# Autodesk Inventor assembly: Intake Full Assembly
(part 2 of 2)
- Mate:580: Intake Roller Plate:1 ↔ COTS_92949A265_1-2in long Stainless Steel Button Head Screw:19
- Mate:581: Intake Roller Plate:1 ↔ COTS_92949A265_1-2in long Stainless Steel Button Head Screw:21
- Mate:582: Intake Roller Plate:1 ↔ COTS_92949A265_1-2in long Stainless Steel Button Head Screw:9
- Mate:583: Intake Roller Plate:1 ↔ COTS_92949A265_1-2in long Stainless Steel Button Head Screw:9
- Mate:584: Intake Roller Plate:1 ↔ COTS_92949A265_1-2in long Stainless Steel Button Head Screw:21
- Mate:585: Intake Roller Plate:1 ↔ COTS_92949A265_1-2in long Stainless Steel Button Head Screw:19
- Mate:586: Intake Roller Plate:1 ↔ COTS_92949A265_1-2in long Stainless Steel Button Head Screw:6
- Mate:587: Intake Roller Plate:1 ↔ COTS_92949A265_1-2in long Stainless Steel Button Head Screw:20
- Mate:588: Intake Roller Plate:1 ↔ COTS_92949A265_1-2in long Stainless Steel Button Head Screw:8
- Mate:589: INTK_001_PulleyCover:1 ↔ COTS_92949A265_1-2in long Stainless Steel Button Head Screw:14
- Mate:590: INTK_001_PulleyCover:1 ↔ COTS_92949A265_1-2in long Stainless Steel Button Head Screw:15
- Mate:591: INTK_001_PulleyCover:1 ↔ COTS_92949A265_1-2in long Stainless Steel Button Head Screw:24
- Mate:592: INTK_001_PulleyCover:1 ↔ COTS_92949A265_1-2in long Stainless Steel Button Head Screw:17
- Mate:593: INTK_001_PulleyCover:1 ↔ COTS_92949A265_1-2in long Stainless Steel Button Head Screw:18
- Mate:594: INTK_001_PulleyCover:1 ↔ COTS_92949A265_1-2in long Stainless Steel Button Head Screw:7
- Mate:595: INTK_001_PulleyCover:1 ↔ COTS_92949A265_1-2in long Stainless Steel Button Head Screw:16
- Mate:596: INTK_001_PulleyCover:2 ↔ COTS_92949A265_1-2in long Stainless Steel Button Head Screw:2
- Mate:597: INTK_001_PulleyCover:2 ↔ COTS_92949A265_1-2in long Stainless Steel Button Head Screw:5
- Mate:598: INTK_001_PulleyCover:2 ↔ COTS_92949A265_1-2in long Stainless Steel Button Head Screw:4
- Mate:599: INTK_001_PulleyCover:2 ↔ COTS_92949A265_1-2in long Stainless Steel Button Head Screw:1
- Mate:600: INTK_001_PulleyCover:2 ↔ COTS_92949A265_1-2in long Stainless Steel Button Head Screw:12
- Mate:601: INTK_001_PulleyCover:2 ↔ COTS_92949A265_1-2in long Stainless Steel Button Head Screw:13
- Mate:602: INTK_001_PulleyCover:2 ↔ COTS_92949A265_1-2in long Stainless Steel Button Head Screw:3
- Mate:603: INTK_001_PulleyCover:2 ↔ COTS_92949A265_1-2in long Stainless Steel Button Head Screw:13
- Mate:604: INTK_001_PulleyCover:2 ↔ COTS_92949A265_1-2in long Stainless Steel Button Head Screw:3
- Mate:605: INTK_001_PulleyCover:2 ↔ COTS_92949A265_1-2in long Stainless Steel Button Head Screw:1
- Mate:606: INTK_001_PulleyCover:2 ↔ COTS_92949A265_1-2in long Stainless Steel Button Head Screw:2
- Mate:607: INTK_001_PulleyCover:2 ↔ COTS_92949A265_1-2in long Stainless Steel Button Head Screw:5
- Mate:608: INTK_001_PulleyCover:2 ↔ COTS_92949A265_1-2in long Stainless Steel Button Head Screw:4
- Mate:609: INTK_001_PulleyCover:2 ↔ COTS_92949A265_1-2in long Stainless Steel Button Head Screw:12
- Mate:610: Intake Roller Plate:2 ↔ COTS_92949A265_1-2in long Stainless Steel Button Head Screw:26
- Mate:611: Intake Roller Plate:2 ↔ COTS_92949A265_1-2in long Stainless Steel Button Head Screw:11
- Mate:612: Intake Roller Plate:2 ↔ COTS_92949A265_1-2in long Stainless Steel Button Head Screw:25
- Mate:613: Intake Roller Plate:2 ↔ COTS_92949A265_1-2in long Stainless Steel Button Head Screw:27
- Mate:614: Intake Roller Plate:2 ↔ COTS_92949A265_1-2in long Stainless Steel Button Head Screw:23
- Mate:615: Intake Roller Plate:2 ↔ COTS_92949A265_1-2in long Stainless Steel Button Head Screw:22
- Mate:616: Intake Roller Plate:2 ↔ COTS_92949A265_1-2in long Stainless Steel Button Head Screw:26
- Mate:617: Intake Roller Plate:2 ↔ COTS_92949A265_1-2in long Stainless Steel Button Head Screw:22
- Mate:618: Intake Roller Plate:2 ↔ COTS_92949A265_1-2in long Stainless Steel Button Head Screw:23
- Mate:619: Intake Roller Plate:2 ↔ COTS_92949A265_1-2in long Stainless Steel Button Head Screw:27
- Mate:620: Intake Roller Plate:2 ↔ COTS_92949A265_1-2in long Stainless Steel Button Head Screw:25
- Mate:621: Intake Roller Plate:2 ↔ COTS_92949A265_1-2in long Stainless Steel Button Head Screw:11
- Mate:622: COTS_217-2592_VersaHub:2 ↔ COTS_91251A196_Black-Oxide Alloy Steel Socket Head Screw_5-8in:3
- Mate:623: COTS_217-2592_VersaHub:2 ↔ COTS_91251A196_Black-Oxide Alloy Steel Socket Head Screw_5-8in:1
- Mate:624: COTS_217-2592_VersaHub:2 ↔ COTS_91251A196_Black-Oxide Alloy Steel Socket Head Screw_5-8in:2
- Mate:625: COTS_217-2592_VersaHub:2 ↔ COTS_91251A196_Black-Oxide Alloy Steel Socket Head Screw_5-8in:11
- Mate:626: COTS_217-2592_VersaHub:2 ↔ COTS_91251A196_Black-Oxide Alloy Steel Socket Head Screw_5-8in:4
- Mate:627: COTS_217-2592_VersaHub:2 ↔ COTS_91251A196_Black-Oxide Alloy Steel Socket Head Screw_5-8in:6
- Mate:628: COTS_217-2592_VersaHub:2 ↔ COTS_91251A196_Black-Oxide Alloy Steel Socket Head Screw_5-8in:4
- Mate:629: COTS_217-2592_VersaHub:2 ↔ COTS_91251A196_Black-Oxide Alloy Steel Socket Head Screw_5-8in:6
- Mate:630: COTS_217-2592_VersaHub:2 ↔ COTS_91251A196_Black-Oxide Alloy Steel Socket Head Screw_5-8in:11
- Mate:631: COTS_217-2592_VersaHub:2 ↔ COTS_91251A196_Black-Oxide Alloy Steel Socket Head Screw_5-8in:2
- Mate:632: COTS_217-2592_VersaHub:2 ↔ COTS_91251A196_Black-Oxide Alloy Steel Socket Head Screw_5-8in:3
- Mate:633: COTS_217-2592_VersaHub:2 ↔ COTS_91251A196_Black-Oxide Alloy Steel Socket Head Screw_5-8in:1
- Mate:634: COTS_217-2592_VersaHub:3 ↔ COTS_91251A196_Black-Oxide Alloy Steel Socket Head Screw_5-8in:12
- Mate:635: COTS_217-2592_VersaHub:3 ↔ COTS_91251A196_Black-Oxide Alloy Steel Socket Head Screw_5-8in:7
- Mate:636: COTS_217-2592_VersaHub:3 ↔ COTS_91251A196_Black-Oxide Alloy Steel Socket Head Screw_5-8in:10
- Mate:637: COTS_217-2592_VersaHub:3 ↔ COTS_91251A196_Black-Oxide Alloy Steel Socket Head Screw_5-8in:9
- Mate:638: COTS_217-2592_VersaHub:3 ↔ COTS_91251A196_Black-Oxide Alloy Steel Socket Head Screw_5-8in:5
- Mate:639: COTS_217-2592_VersaHub:3 ↔ COTS_91251A196_Black-Oxide Alloy Steel Socket Head Screw_5-8in:8
- Mate:640: COTS_217-2592_VersaHub:3 ↔ COTS_91251A196_Black-Oxide Alloy Steel Socket Head Screw_5-8in:12
- Mate:641: COTS_217-2592_VersaHub:3 ↔ COTS_91251A196_Black-Oxide Alloy Steel Socket Head Screw_5-8in:7
- Mate:642: COTS_217-2592_VersaHub:3 ↔ COTS_91251A196_Black-Oxide Alloy Steel Socket Head Screw_5-8in:10
- Mate:643: COTS_217-2592_VersaHub:3 ↔ COTS_91251A196_Black-Oxide Alloy Steel Socket Head Screw_5-8in:8
- Mate:644: COTS_217-2592_VersaHub:3 ↔ COTS_91251A196_Black-Oxide Alloy Steel Socket Head Screw_5-8in:5
- Mate:645: COTS_217-2592_VersaHub:3 ↔ COTS_91251A196_Black-Oxide Alloy Steel Socket Head Screw_5-8in:9
- Mate:646: COTS_91251A196_Black-Oxide Alloy Steel Socket Head Screw_5-8in:10 ↔ COTS_90631A009_8-32_Low-Strength Steel Nylon-Insert Locknut:11
- Mate:647: Intake Roller Plate:2 ↔ COTS_90631A009_8-32_Low-Strength Steel Nylon-Insert Locknut:11
- Mate:648: COTS_91251A196_Black-Oxide Alloy Steel Socket Head Screw_5-8in:8 ↔ COTS_90631A009_8-32_Low-Strength Steel Nylon-Insert Locknut:1
- Mate:649: Intake Roller Plate:2 ↔ COTS_90631A009_8-32_Low-Strength Steel Nylon-Insert Locknut:1
- Mate:650: COTS_91251A196_Black-Oxide Alloy Steel Socket Head Screw_5-8in:7 ↔ COTS_90631A009_8-32_Low-Strength Steel Nylon-Insert Locknut:12
- Mate:651: Intake Roller Plate:2 ↔ COTS_90631A009_8-32_Low-Strength Steel Nylon-Insert Locknut:12
- Mate:652: COTS_91251A196_Black-Oxide Alloy Steel Socket Head Screw_5-8in:12 ↔ COTS_90631A009_8-32_Low-Strength Steel Nylon-Insert Locknut:4
- Mate:653: Intake Roller Plate:2 ↔ COTS_90631A009_8-32_Low-Strength Steel Nylon-Insert Locknut:4
- Mate:654: COTS_91251A196_Black-Oxide Alloy Steel Socket Head Screw_5-8in:5 ↔ COTS_90631A009_8-32_Low-Strength Steel Nylon-Insert Locknut:8
- Mate:655: Intake Roller Plate:2 ↔ COTS_90631A009_8-32_Low-Strength Steel Nylon-Insert Locknut:8
- Mate:656: COTS_91251A196_Black-Oxide Alloy Steel Socket Head Screw_5-8in:9 ↔ COTS_90631A009_8-32_Low-Strength Steel Nylon-Insert Locknut:7
- Mate:657: Intake Roller Plate:2 ↔ COTS_90631A009_8-32_Low-Strength Steel Nylon-Insert Locknut:7
- Mate:658: COTS_91251A196_Black-Oxide Alloy Steel Socket Head Screw_5-8in:3 ↔ COTS_90631A009_8-32_Low-Strength Steel Nylon-Insert Locknut:5
- Mate:659: COTS_91251A196_Black-Oxide Alloy Steel Socket Head Screw_5-8in:2 ↔ COTS_90631A009_8-32_Low-Strength Steel Nylon-Insert Locknut:9
- Mate:660: COTS_91251A196_Black-Oxide Alloy Steel Socket Head Screw_5-8in:4 ↔ COTS_90631A009_8-32_Low-Strength Steel Nylon-Insert Locknut:10
- Mate:661: COTS_91251A196_Black-Oxide Alloy Steel Socket Head Screw_5-8in:6 ↔ COTS_90631A009_8-32_Low-Strength Steel Nylon-Insert Locknut:6
- Mate:662: COTS_91251A196_Black-Oxide Alloy Steel Socket Head Screw_5-8in:11 ↔ COTS_90631A009_8-32_Low-Strength Steel Nylon-Insert Locknut:2
- Mate:663: COTS_91251A196_Black-Oxide Alloy Steel Socket Head Screw_5-8in:1 ↔ COTS_90631A009_8-32_Low-Strength Steel Nylon-Insert Locknut:3
- Mate:664: Intake Roller Plate:1 ↔ COTS_90631A009_8-32_Low-Strength Steel Nylon-Insert Locknut:3
- Mate:665: Intake Roller Plate:1 ↔ COTS_90631A009_8-32_Low-Strength Steel Nylon-Insert Locknut:5
- Mate:666: Intake Roller Plate:1 ↔ COTS_90631A009_8-32_Low-Strength Steel Nylon-Insert Locknut:9
- Mate:667: Intake Roller Plate:1 ↔ COTS_90631A009_8-32_Low-Strength Steel Nylon-Insert Locknut:10
- Mate:668: Intake Roller Plate:1 ↔ COTS_90631A009_8-32_Low-Strength Steel Nylon-Insert Locknut:6
- Mate:669: Intake Roller Plate:1 ↔ COTS_90631A009_8-32_Low-Strength Steel Nylon-Insert Locknut:2
- Mate:670: Intake Roller Plate:1 ↔ COTS_92949A265_1-2in long Stainless Steel Button Head Screw:28
- Mate:674: Intake Roller Plate:1 ↔ COTS_92949A265_1-2in long Stainless Steel Button Head Screw:28
- Mate:675: COTS_WCP-0783_1.125ODHexBearing:19 ↔ INtk_010_Belt2:1
- Mate:676 (0.508 mm): COTS_WCP-0783_1.125ODHexBearing:14 ↔ INtk_010_Belt2:1
- Mate:677: COTS_HTD5M10mm15T_WCP-1420:4 ↔ INtk_010_Belt2:1
- Mate:678: COTS_WCP-0783_1.125ODHexBearing:14 ↔ INTK_009_Belt1:1
- Mate:679: INTK_006_Spacer6:1 ↔ INTK_009_Belt1:1
- Mate:680: COTW_HTD5M10mm12T_WCP-0076:1 ↔ INTK_009_Belt1:1
- Mate:681: COTS_WCP-0783_1.125ODHexBearing:20 ↔ INtk_010_Belt2:2
- Mate:682: COTS_WCP-0783_1.125ODHexBearing:15 ↔ INtk_010_Belt2:2
- Mate:683: COTS_HTD5M10mm15T_WCP-1420:1 ↔ INtk_010_Belt2:2
- Mate:684: COTS_WCP-0799_0.5inchHexShaftCollar:8 ↔ INTK_011_Belt3:1
- Mate:685: COTS_WCP-0799_0.5inchHexShaftCollar:7 ↔ INTK_011_Belt3:1
- Mate:686: COTS_HTD5M10mm18T_WCP-0563:18 ↔ INTK_011_Belt3:1
- Mate:687: COTS_WCP-0799_0.5inchHexShaftCollar:6 ↔ INTK_011_Belt3:2
- Mate:688: COTS_WCP-0799_0.5inchHexShaftCollar:5 ↔ INTK_011_Belt3:2
- Mate:689: COTS_HTD5M10mm18T_WCP-0563:5 ↔ INTK_011_Belt3:2
- Mate:690: COTS_WCP-0799_0.5inchHexShaftCollar:11 ↔ INTK_012_Belt4:1
- Mate:691: COTS_WCP-0799_0.5inchHexShaftCollar:9 ↔ INTK_012_Belt4:1
- Mate:692: COTS_HTD5M10mm18T_WCP-0563:4 ↔ INTK_012_Belt4:1
- Mate:693: COTS_WCP-0799_0.5inchHexShaftCollar:10 ↔ INTK_012_Belt4:2
- Mate:694: COTS_WCP-0799_0.5inchHexShaftCollar:12 ↔ INTK_012_Belt4:2
- Mate:695: Intake Roller Plate:2 ↔ INTK_012_Belt4:2
- Mate:696: INTK_005_Spacer5:6 ↔ INTK_013_Belt5:1
- Mate:697: INTK_005_Spacer5:7 ↔ INTK_013_Belt5:1
- Mate:698: COTS_HTD5M10mm18T_WCP-0563:15 ↔ INTK_013_Belt5:1
- Mate:699: INTK_005_Spacer5:4 ↔ INTK_013_Belt5:2
- Mate:700: INTK_005_Spacer5:2 ↔ INTK_013_Belt5:2
- Mate:701: COTS_HTD5M10mm18T_WCP-0563:11 ↔ INTK_013_Belt5:2
- Mate:702: INTK_005_Spacer5:3 ↔ INTK_014_Belt6:1
- Mate:703: COTS_WCP-0783_1.125ODHexBearing:17 ↔ INTK_014_Belt6:1
- Mate:704: COTS_HTD5M10mm18T_WCP-0563:1 ↔ INTK_014_Belt6:1
- Mate:705: Intake Roller Plate:1 ↔ COTS_92949A265_1-2in long Stainless Steel Button Head Screw:29
- Mate:706: Intake Roller Plate:1 ↔ COTS_92949A265_1-2in long Stainless Steel Button Head Screw:29
- Mate:707: COTS_REV-21-1650-V1.1:2 ↔ INTK_015_Spacer8:1
- Mate:708: COTS_REV-21-1650-V1.1:2 ↔ INTK_015_Spacer8:1
